# Autodesk Inventor assembly: syringeAssem
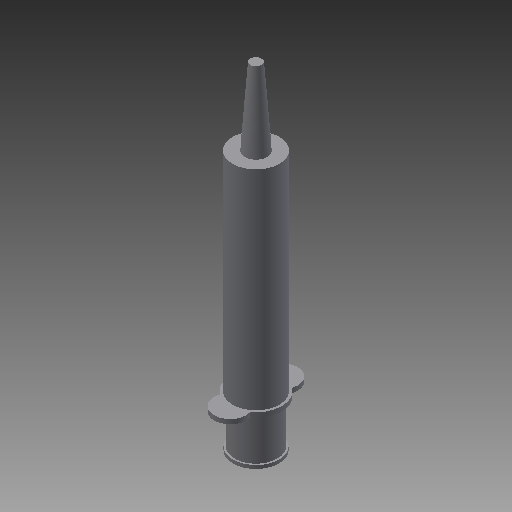
[picture p0: Inventor's stored thumbnail of the model, 512x512]
Saved by Autodesk Inventor 2018 (Build 220112000, 112)
## iProperties
Created: 2020-03-06
Part Number: syringeAssem
Document SubType Name: Assembly
Designer: Jesse R-B
Author: Jesse R-B
## Documents named in this file (3)
- C:\Users\Jesse R-B\Documents\Inventor\400\V2\syringeAssem.iam
- C:\Users\Jesse R-B\Documents\Inventor\400\V2\syringe.ipt
- C:\Users\Jesse R-B\Documents\Inventor\400\V2\plunger.ipt
## Components (2 placed, 2 different names)
1. syringe:1 — Mate:1
2. plunger:1 — Mate:1
## Relationships (1: Mate 1)
- Mate:1: syringe:1 ↔ plunger:1
